# Autodesk Inventor assembly: PLA-shaft-coupler
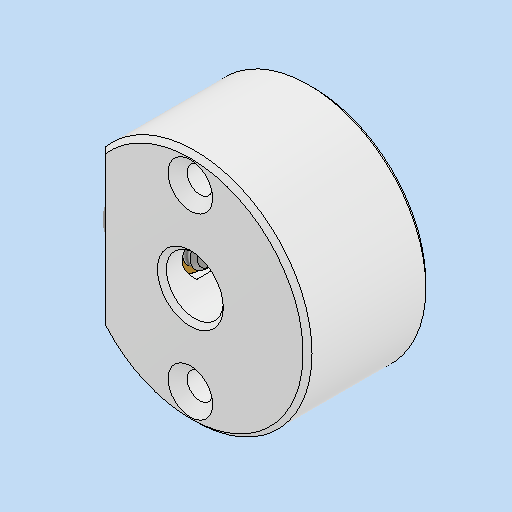
[picture p0: Inventor's stored thumbnail of the model, 512x512]
Saved by Autodesk Inventor 2025 (Build 290162000, 162)
## iProperties
Created: 2025-05-29
Part Number: PLA-shaft-coupler
Document SubType Name: Assembly
Designer: kuzmin
Author: kuzmin
## Documents named in this file (4)
- C:\Users\queez\Dropbox\Drawings\PIHTI\LIBS\PLA-shaft-coupler.iam
- C:\Users\queez\Dropbox\Drawings\PIHTI\LIBS\shaft-coupler-pla.ipt
- C:\Users\queez\Dropbox\Drawings\PIHTI\ContentCenter\Fastners\brass-insert-m3x5.ipt
- C:\Users\queez\Dropbox\Drawings\PIHTI\ContentCenter\Fastners\M3x6-BHCS.ipt
## Components (3 placed, 3 different names)
1. shaft-coupler-pla:1
2. brass-insert-m3x5:1
3. Broached Hexagon Socket Button Head Cap Screw - Metric M3 x 0.5 x 6:1
## Relationships (2: RevoluteJoint 2)
- [RevoluteJoint]: shaft-coupler-pla:1 ↔ brass-insert-m3x5:1
- [RevoluteJoint]: brass-insert-m3x5:1 ↔ Broached Hexagon Socket Button Head Cap Screw - Metric M3 x 0.5 x 6:1
